# Autodesk Inventor assembly: LongCap
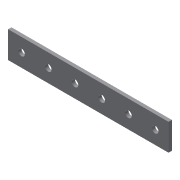
[picture p0: Inventor's stored thumbnail of the model, 180x180]
Saved by Autodesk Inventor 2015 (Build 190159000, 159)
## iProperties
Created: 2015-03-09
Part Number: LongCap
Document SubType Name: Assembly
Designer: Jaden
Author: Jaden
## Documents named in this file (2)
- E:\ReDesign\LongCap.iam
- E:\ReDesign\Imported Components\Endcap\Endcap.ipt
## Components (6 placed, 1 different names)
1. Endcap:1 — Mate:11, Mate:12
2. Endcap:2 — Mate:9, Mate:10, Mate:11, Mate:12
3. Endcap:3 — Mate:2, Mate:3, Mate:4, Mate:7, Mate:8
4. Endcap:4 — Mate:7, Mate:8, Mate:9, Mate:10
5. Endcap:5 — Mate:1, Mate:5, Mate:6
6. Endcap:6 — Mate:1, Mate:2, Mate:3, Mate:4, Mate:5, Mate:6
## Relationships (12: Mate 12)
- Mate:1: Endcap:5 ↔ Endcap:6
- Mate:2: Endcap:3 ↔ Endcap:6
- Mate:3: Endcap:3 ↔ Endcap:6
- Mate:4: Endcap:3 ↔ Endcap:6
- Mate:5: Endcap:5 ↔ Endcap:6
- Mate:6: Endcap:5 ↔ Endcap:6
- Mate:7: Endcap:3 ↔ Endcap:4
- Mate:8: Endcap:3 ↔ Endcap:4
- Mate:9: Endcap:2 ↔ Endcap:4
- Mate:10: Endcap:2 ↔ Endcap:4
- Mate:11: Endcap:1 ↔ Endcap:2
- Mate:12: Endcap:1 ↔ Endcap:2
